# Autodesk Inventor assembly: FE-00002-12
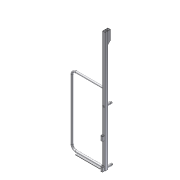
[picture p0: Inventor's stored thumbnail of the model, 180x180]
Saved by Autodesk Inventor 2012 (Build 160160000, 160)
## iProperties
Created: 2008-05-15
Part Number: FE-00002-12
Document SubType Name: Assembly
Designer: narosenberg
Author: narosenberg
## Documents named in this file (8)
- C:\Data Folder\FRC 2012 Field\Components\FE-00002-12.iam
- C:\Data Folder\FRC 2012 Field\Components\FE-00002-03.ipt
- C:\Data Folder\FRC 2012 Field\Components\FE-00002-05.ipt
- C:\Data Folder\FRC 2012 Field\Components\FE-00002-06.ipt
- C:\Data Folder\FRC 2012 Field\Components\FE-00002-01.ipt
- C:\Data Folder\FRC 2012 Field\Components\FE-00002-02.ipt
- C:\Data Folder\FRC 2012 Field\Components\FE-00002-09.ipt
- C:\Data Folder\FRC 2012 Field\Components\FE-00002-07.ipt
## Components (8 placed, 7 different names)
1. FE-00002-06:1 — Mate:15, Mate:16, Tangent:3, Angle:2, Flush:5, Mate:17
2. FE-00002-07:1 — Mate:16, Tangent:3, Angle:2, Flush:5, Mate:18, Flush:6
3. FE-00002-05:1 — Flush:3, Insert:1, Insert:2, Mate:6, Mate:7, Mate:8, Mate:9, Tangent:2, Flush:4, Mate:17, Flush:6
4. FE-00002-01:1 — Insert:1
5. FE-00002-02:1 — Insert:2
6. FE-00002-03:1 — Mate:6, Mate:7
7. FE-00002-09:1 — Mate:12, Tangent:2, Flush:4, Insert:3
8. FE-00002-09:2 — Mate:13, Insert:3
## Relationships (26: Mate 15, Flush 4, Insert 3, Angle 2, Tangent 2)
- Mate:2
- Angle:1 (90 deg)
- Flush:3 (-22.225 mm): FE-00002-05:1
- Mate:5
- Insert:1: FE-00002-05:1 ↔ FE-00002-01:1
- Insert:2: FE-00002-05:1 ↔ FE-00002-02:1
- Mate:6: FE-00002-05:1 ↔ FE-00002-03:1
- Mate:7: FE-00002-05:1 ↔ FE-00002-03:1
- Mate:8: FE-00002-05:1
- Mate:9: FE-00002-05:1
- Mate:10
- Mate:11
- Mate:12: FE-00002-09:1
- Mate:13: FE-00002-09:2
- Mate:14
- Tangent:2: FE-00002-05:1 ↔ FE-00002-09:1
- Flush:4: FE-00002-05:1 ↔ FE-00002-09:1
- Insert:3 (441.325 mm): FE-00002-09:1 ↔ FE-00002-09:2
- Mate:15: FE-00002-06:1
- Mate:16: FE-00002-06:1 ↔ FE-00002-07:1
- Tangent:3: FE-00002-06:1 ↔ FE-00002-07:1
- Angle:2 (0 deg): FE-00002-06:1 ↔ FE-00002-07:1
- Flush:5 (-25.4 mm): FE-00002-06:1 ↔ FE-00002-07:1
- Mate:17: FE-00002-06:1 ↔ FE-00002-05:1
- Mate:18: FE-00002-07:1
- Flush:6: FE-00002-07:1 ↔ FE-00002-05:1
